# Autodesk Inventor assembly: Stół
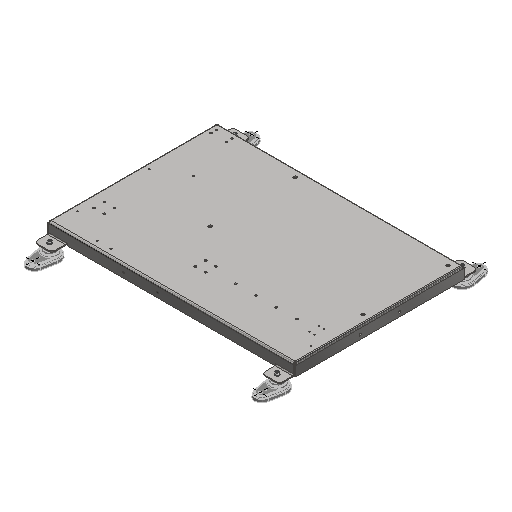
[picture p0: Inventor's stored thumbnail of the model, 512x512]
Saved by Autodesk Inventor 2024.3 (Build 283343000, 343)
## iProperties
Created: 2025-06-06
Part Number: Stół
Document SubType Name: Assembly
Designer: MPA
Author: MPA
## Documents named in this file (5)
- C:\MPA - shortPath\magisterka\V3\Workspace\Stół.iam
- C:\MPA - shortPath\magisterka\V3\Workspace\Stół.ipt
- C:\MPA - shortPath\magisterka\V3\Workspace\Zakupowe\LV_FO-60-14_SJF-M6_0\LV_FO-60-14_SJF-M6_0\LV_FO-60-14_SJF-M6_0.iam
- C:\MPA - shortPath\magisterka\V3\Workspace\cc\en-US\DIN 125-1  A\DIN 125 - A 6,4.ipt
- C:\MPA - shortPath\magisterka\V3\Workspace\cc\en-US\DIN 912\DIN 912 - M6 x 1 x 12 x 9,5.ipt
## Components (13 placed, 4 different names)
1. Stół:1 — Flush:1, Flush:2, Flush:3, Insert:1, Angle:1, Mate:1, Mate:2
2. LV_FO-60-14_SJF-M6_0:1 [sub-assembly] — Insert:1, Angle:1
3. DIN 125-1 A A 6,4:1 — Mate:1, Mate:2, Insert:2
4. DIN 912 - replaced by DIN EN ISO 4762 M6 x 12:1 — Insert:2
5. LV_FO-60-14_SJF-M6_0:2 [sub-assembly]
6. LV_FO-60-14_SJF-M6_0:3 [sub-assembly]
7. LV_FO-60-14_SJF-M6_0:4 [sub-assembly]
8. DIN 125-1 A A 6,4:2
9. DIN 912 - replaced by DIN EN ISO 4762 M6 x 12:2
10. DIN 125-1 A A 6,4:3
11. DIN 912 - replaced by DIN EN ISO 4762 M6 x 12:3
12. DIN 125-1 A A 6,4:4
13. DIN 912 - replaced by DIN EN ISO 4762 M6 x 12:4
## Relationships (8: Flush 3, Insert 2, Mate 2, Angle 1)
- Flush:1: Stół:1
- Flush:2: Stół:1
- Flush:3: Stół:1
- Insert:1: Stół:1 ↔ LV_FO-60-14_SJF-M6_0:1
- Angle:1 (0 deg): Stół:1 ↔ LV_FO-60-14_SJF-M6_0:1
- Mate:1: Stół:1 ↔ DIN 125-1 A A 6,4:1
- Mate:2: Stół:1 ↔ DIN 125-1 A A 6,4:1
- Insert:2: DIN 125-1 A A 6,4:1 ↔ DIN 912 - replaced by DIN EN ISO 4762 M6 x 12:1
